# Autodesk Inventor assembly: ASY SLM 1650 filter-distribution-system 1000
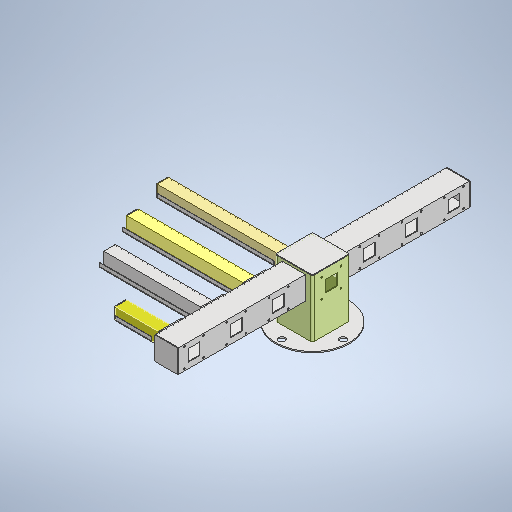
[picture p0: Inventor's stored thumbnail of the model, 512x512]
Saved by Autodesk Inventor 2025.4 (Build 294407000, 407)
## iProperties
Created: 2025-06-24
Part Number: ASY SLM 1650 filter-distribution-system 1000
Document SubType Name: Assembly
Designer: admin
Author: user
## Documents named in this file (15)
- C:\Users\admin\Documents\Inventor\NDA-Nyyda\ASY PNS 1650 filter-distribution-system 1000.iam
- C:\Users\admin\Documents\Inventor\NDA-Nyyda\PNS 169859 DIM filter-distribution-system 1000.ipt
- C:\Users\admin\Documents\Inventor\NDA-Nyyda\PNS 1651 FDS MAIN  FLANGE.ipt
- C:\Users\admin\Documents\Inventor\NDA-Nyyda\PNS 1652 FDS Central tube wall.ipt
- C:\Users\admin\Documents\Inventor\NDA-Nyyda\ASY PNS FDS way1_1600.iam
- C:\Users\admin\Documents\Inventor\NDA-Nyyda\ASY PNS 1662 FDS way 2.iam
- C:\Users\admin\Documents\Inventor\NDA-Nyyda\ASY PNS FDS way3_1600.iam
- C:\Users\admin\Documents\Inventor\NDA-Nyyda\PNS 1665 FDS 1000 CUP 1.ipt
- C:\Users\admin\Documents\Inventor\NDA-Nyyda\SLM 1424 FDS diam way cup.ipt
- C:\Users\admin\Documents\Inventor\NDA-Nyyda\SLM 1421 FDS Diam way flange 1.ipt
- C:\Users\admin\Documents\Inventor\NDA-Nyyda\NDA-1661 (fds) main way tube.ipt
- C:\Users\admin\Documents\Inventor\NDA-Nyyda\NDA-514 roof 4.ipt
- C:\Users\admin\Documents\Inventor\NDA-Nyyda\SLM 1425 FDS Way FLANGE.ipt
- C:\Users\admin\Documents\Inventor\NDA-Nyyda\NDA-1662 FDS 1000 way tube 4.ipt
- C:\Users\admin\Documents\Inventor\NDA-Nyyda\NDA-513 roof 4.ipt
## Components (17 placed, 14 different names)
1. PNS 169859 DIM filter-distribution-system 1000.ipt:1 — Mate:5, Mate:4
2. PNS 1651 FDS MAIN  FLANGE.ipt:1 — Flush:1, Mate:5, Flush:5, Flush:6
3. PNS 1652 FDS Central tube wall.ipt:1 — Flush:1, Flush:4, Flush:3, Mate:6, Rigid:1, Flush:6, Rigid:5
4. PNS 1652 FDS Central tube wall.ipt:2 — Rigid:1, Mate:5, Flush:5, Rigid:2, Rigid:6
5. ASY PNS FDS way1_1600.iam:3 [sub-assembly] — Rigid:6
6. ASY PNS 1662 FDS way 2.iam:4 [sub-assembly] — Rigid:10
7. ASY PNS FDS way3_1600.iam:3 [sub-assembly] — Rigid:9, Rigid:11
8. PNS 1665 FDS 1000 CUP 1.ipt:1 — Flush:4, Flush:3, Mate:6
9. SLM 1424 FDS diam way cup:1 — Rigid:3
10. SLM 1421 FDS Diam way flange 1:1
11. NDA-1661 (fds) main way tube:1 — Rigid:2, Rigid:3
12. SLM 1424 FDS diam way cup:3
13. NDA-1661 (fds) main way tube:2 — Rigid:5, Rigid:10, Rigid:11, Rigid:14
14. NDA-514 roof 4:1 — Rigid:9
15. SLM 1425 FDS Way FLANGE:1 — Rigid:13, Rigid:14
16. NDA-1662 FDS 1000 way tube 4:1 — Rigid:12, Rigid:13
17. NDA-513 roof 4:1 — Rigid:12
## Relationships (21: WeldJoint 12, Flush 5, Mate 4)
- Mate:5: PNS 169859 DIM filter-distribution-system 1000.ipt:1
- Mate:4: PNS 169859 DIM filter-distribution-system 1000.ipt:1
- Flush:1: PNS 1651 FDS MAIN  FLANGE.ipt:1 ↔ PNS 1652 FDS Central tube wall.ipt:1
- Flush:4: PNS 1652 FDS Central tube wall.ipt:1 ↔ PNS 1665 FDS 1000 CUP 1.ipt:1
- Flush:3: PNS 1652 FDS Central tube wall.ipt:1 ↔ PNS 1665 FDS 1000 CUP 1.ipt:1
- Mate:6: PNS 1652 FDS Central tube wall.ipt:1 ↔ PNS 1665 FDS 1000 CUP 1.ipt:1
- Rigid:1 [WeldJoint]: PNS 1652 FDS Central tube wall.ipt:1 ↔ PNS 1652 FDS Central tube wall.ipt:2
- Mate:5: PNS 1651 FDS MAIN  FLANGE.ipt:1 ↔ PNS 1652 FDS Central tube wall.ipt:2
- Flush:5: PNS 1651 FDS MAIN  FLANGE.ipt:1 ↔ PNS 1652 FDS Central tube wall.ipt:2
- Flush:6: PNS 1651 FDS MAIN  FLANGE.ipt:1 ↔ PNS 1652 FDS Central tube wall.ipt:1
- Rigid:2 [WeldJoint]: PNS 1652 FDS Central tube wall.ipt:2 ↔ NDA-1661 (fds) main way tube:1
- Rigid:3 [WeldJoint]: SLM 1424 FDS diam way cup:1 ↔ NDA-1661 (fds) main way tube:1
- [WeldJoint]: SLM 1424 FDS diam way cup:3 ↔ NDA-1661 (fds) main way tube:2
- Rigid:5 [WeldJoint]: PNS 1652 FDS Central tube wall.ipt:1 ↔ NDA-1661 (fds) main way tube:2
- Rigid:6 [WeldJoint]: PNS 1652 FDS Central tube wall.ipt:2 ↔ ASY PNS FDS way1_1600.iam:3
- Rigid:9 [WeldJoint]: ASY PNS FDS way3_1600.iam:3 ↔ NDA-514 roof 4:1
- Rigid:10 [WeldJoint]: ASY PNS 1662 FDS way 2.iam:4 ↔ NDA-1661 (fds) main way tube:2
- Rigid:11 [WeldJoint]: ASY PNS FDS way3_1600.iam:3 ↔ NDA-1661 (fds) main way tube:2
- Rigid:12 [WeldJoint]: NDA-1662 FDS 1000 way tube 4:1 ↔ NDA-513 roof 4:1
- Rigid:13 [WeldJoint]: SLM 1425 FDS Way FLANGE:1 ↔ NDA-1662 FDS 1000 way tube 4:1
- Rigid:14 [WeldJoint]: NDA-1661 (fds) main way tube:2 ↔ SLM 1425 FDS Way FLANGE:1
## Named parameters: d68_d67 = 0 mm
